# Autodesk Inventor assembly: AssemblyV3
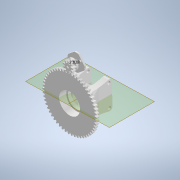
[picture p0: Inventor's stored thumbnail of the model, 180x180]
Saved by Autodesk Inventor 2022 (Build 260153070, 153G)
## iProperties
Created: 2021-11-03
Part Number: AssemblyV3
Document SubType Name: Assembly
Designer: a laptop
Author: a laptop
## Documents named in this file (7)
- C:\Users\a laptop\Desktop\SumoBot\sumobotLIDAR\AssemblyV3.iam
- C:\Users\a laptop\Desktop\SumoBot\sumobotLIDAR\AssemblyV3\Design Accelerator\Spur Gears1.iam
- C:\Users\a laptop\Desktop\SumoBot\sumobotLIDAR\BigGear54T.ipt
- C:\Users\a laptop\Desktop\SumoBot\sumobotLIDAR\SmallGear9T.ipt
- C:\Users\a laptop\Desktop\SumoBot\sumobotLIDAR\REF_PART\VL53L1X board.ipt
- C:\Users\a laptop\Desktop\SumoBot\sumobotLIDAR\REF_PART\Magnet.ipt
- C:\Users\a laptop\Desktop\SumoBot\sumobotLIDAR\REF_PART\AS5600.ipt
## Components (6 placed, 6 different names)
1. Spur Gears:1 [sub-assembly]
2. BigGear54T:1 — Mate:1, Rotation:1, Mate:3, Angle:2, Flush:1, Angle:3, Flush:2, Mate:4, Mate:5
3. SmallGear9T:1 — Mate:1, Rotation:1, Mate:2, Angle:1, Flush:1, Mate:6, Mate:7
4. VL53L1X board:1 — Angle:3, Flush:2, Mate:4, Mate:5
5. Magnet:1 — Mate:6, Mate:7, Mate:8, Mate:9
6. AS5600:1 — Mate:8, Mate:9
## Relationships (15: Mate 9, Angle 3, Flush 2, RelateRotation 1)
- Mate:1 (32.308 mm): BigGear54T:1 ↔ SmallGear9T:1
- Rotation:1 [RelateRotation] (6 ul): BigGear54T:1 ↔ SmallGear9T:1
- Mate:2: SmallGear9T:1
- Angle:1 (0 deg): SmallGear9T:1
- Mate:3: BigGear54T:1
- Angle:2 (0 deg): BigGear54T:1
- Flush:1: BigGear54T:1 ↔ SmallGear9T:1
- Angle:3 (0 deg): BigGear54T:1 ↔ VL53L1X board:1
- Flush:2: BigGear54T:1 ↔ VL53L1X board:1
- Mate:4: BigGear54T:1 ↔ VL53L1X board:1
- Mate:5 (-35 mm): BigGear54T:1 ↔ VL53L1X board:1
- Mate:6: SmallGear9T:1 ↔ Magnet:1
- Mate:7: SmallGear9T:1 ↔ Magnet:1
- Mate:8: Magnet:1 ↔ AS5600:1
- Mate:9 (0.5 mm): Magnet:1 ↔ AS5600:1
